# Autodesk Inventor assembly: BSHKSA6904ZZ-40_right
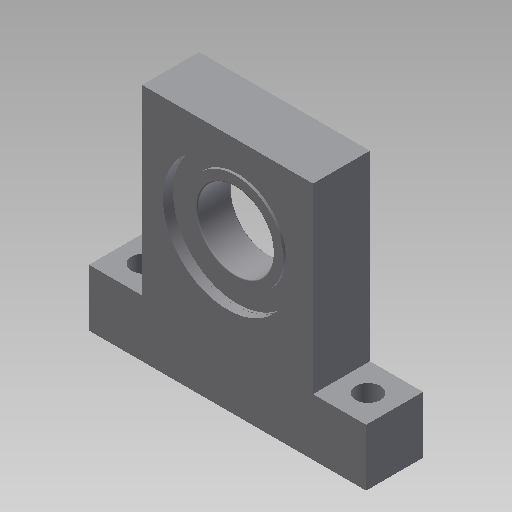
[picture p0: Inventor's stored thumbnail of the model, 512x512]
Saved by Autodesk Inventor 2021.2 (Build 252289000, 289)
## iProperties
Category: PARTsolutions
Company: MISUMI
Part Number: BSHKSA6904ZZ-40_right
Catalog Web Link: www.cadenas.de
Description: BSHKB, BSHK, BSHKA, BSHKSA, BSHFB, BSHF-Bearings with Housings - with Positioning Groove - T-Shaped - Base Face Type
Vendor: MISUMI
Document SubType Name: Assembly
Designer: gisen
Manufacturer: MISUMI
Mass: 38.5292 g
Surface Area: 155.893 cm^2
Volume: 38.5292 cm^3
Density: 1 g/cm^3
Title: BSHKSA6904ZZ-40
Author: Cadenas PARTsolutions
Comments: Bearings with Housings - with Positioning Groove - T-Shaped - Base Face Type
PSOL_IDENT_0: {$CADENAS_DATA\23d-libs\misumi\metric\12_bearing_holders\bshkb_asmtab.prj},259 {VTYP=3D},{STYP=ASSTA
PSOL_IDENT_1: B},{NB=BSHKSA6904ZZ-40},{LINA=BSHKSA6904ZZ-40},{NN=BSHKB, BSHK, BSHKA, BSHKSA, BSHFB, BSHF},{DATE=03
PSOL_IDENT_2: .06.2021 05:36:04},{GEOMDATE=10.09.2019 05:26:06},{VERSION=},{LINEID=210},{WBVAR=TS,MATB,MATH,STH,SE
PSOL_IDENT_3: AL,HH,ALT1,ALT2,ALT3},{WBNUMERIC=HH}  {NB=BSHKSA6904ZZ-40},{LINA=BSHKSA6904ZZ-40},{KT=DUMMY},{PN=BSH
PSOL_IDENT_4: KSA6904ZZ-40},{TYPE=BSHKSA},{TS=HS},{TSALG= 'HS', 'Height h Selectable', 'HC', 'Height h Specified'
PSOL_IDENT_5: },{MATB=SST},{MATBALG= 'ST','Steel','SST','Stainless Steel' },{MATH=A2000},{MATH1= 'A2000','2017 Alu
PSOL_IDENT_6: minum Alloy' },{STH=CA},{STH1=   'CA','Clear Anodizing'     },{ARR=304 Stainless Steel},{BN=6904},{B
PSOL_IDENT_7: N2=6904},{SEAL=ZZ},{SEALALG= 'ZZ', 'ZZ(Double Shielded)', 'VV', 'VV(Non-contact Rubber Seal)', 'DD'
PSOL_IDENT_8: , 'DD(Contact Rubber Seal)' },{HH=40},{HH1=40,50,60},{HH2=[30:80/1]},{DD=20},{D=37},{D3=39.800},{BT=
PSOL_IDENT_9: 1.600},{DDHH=34},{B=9},{H=63},{HD1=23},{L=73},{L1=59},{L2=45},{L3=36.5},{T=15},{S=15},{DD1=6.5},{TEM
PSOL_IDENT_10: P1=2},{NR=},{HHALG=40,50,60},{ALT1=},{ALT1ALG= '', 'Bearing and Retaining Ring Assembled', 'NA'  , '
PSOL_IDENT_11: with NA (Bearing and Retaining Ring not Assembled)'},{ALT1PN=},{ALT2=},{ALT2ALG='', 'w/o Chamfering'
PSOL_IDENT_12: , 'KCC', 'with KCC (C2 Chamfering)'},{ALT2PN=},{BNHALG=2},{ALT3=},{ALT3ALG= '','Not applicable' },{A
PSOL_IDENT_13: LT3PN=},{KKC=10},{PPATH=bshkb/bshkb_temp.prj}
NB: BSHKSA6904ZZ-40
NN: BSHKB, BSHK, BSHKA, BSHKSA, BSHFB, BSHF
NT: Bearings with Housings - with Positioning Groove - T-Shaped - Base Face Type
NBSYN: $PN.
LINA: BSHKSA6904ZZ-40
CATALOG: Misumi
PN: BSHKSA6904ZZ-40
TS: Height h Selectable
MATB: Stainless Steel
MATH: 2017 Aluminum Alloy
STH: Clear Anodizing
ARR: 304 Stainless Steel
BN: 6904
SEAL: ZZ(Double Shielded)
HH: 40
DD: 20
D: 37
DDHH: 34
B: 9
H: 63
L: 73
L1: 59
L2: 45
L3: 36.5
T: 15
S: 15
DD1: 6.5
ALT1: Bearing and Retaining Ring Assembled
ALT2: w/o Chamfering
ALT3: Not applicable
SUPPLIER: MISUMI
ARTICLENO: BSHKSA6904ZZ-40
BOMINFO: BSHKSA6904ZZ-40
CREATOR: CADENAS GmbH
## Documents named in this file (4)
- C:\Users\gisen\workspace\beetle_inventor_model\suspension\BSHKSA6904ZZ-40\BSHKSA6904ZZ-40_right.iam
- C:\Users\gisen\workspace\beetle_inventor_model\suspension\BSHKSA6904ZZ-40\BSHKSA6904ZZ-40_h_right.ipt
- C:\Users\gisen\workspace\beetle_inventor_model\suspension\BSHKSA6904ZZ-40\bearing_6904_right.ipt
- C:\Users\gisen\workspace\beetle_inventor_model\suspension\BSHKSA6904ZZ-40\RRING-C-INT-37_right.ipt
## Components (3 placed, 1 different names)
1. Part1:1 — to_bearing_Z@1 <-> to_housing_Z@2, to_bearing_XY@1 <-> to_housing_XY@2, to_rring_Z@1 <-> rr_Z@3, to_rring_XY@1 <-> rr_XY@3, to_bearing_YZ@1 <-> to_housing_YZ@2, to_rring_YZ@1 <-> rr_YZ@3
2. Part1:2 — to_bearing_Z@1 <-> to_housing_Z@2, to_bearing_XY@1 <-> to_housing_XY@2, to_bearing_YZ@1 <-> to_housing_YZ@2
3. Part1:3 — to_rring_Z@1 <-> rr_Z@3, to_rring_XY@1 <-> rr_XY@3, to_rring_YZ@1 <-> rr_YZ@3
## Relationships (6: Mate 4, Angle 2)
- to_bearing_Z@1 <-> to_housing_Z@2 [Mate]: Part1:1 ↔ Part1:2
- to_bearing_XY@1 <-> to_housing_XY@2 [Mate] (-9 mm): Part1:1 ↔ Part1:2
- to_rring_Z@1 <-> rr_Z@3 [Mate]: Part1:1 ↔ Part1:3
- to_rring_XY@1 <-> rr_XY@3 [Mate]: Part1:1 ↔ Part1:3
- to_bearing_YZ@1 <-> to_housing_YZ@2 [Angle] (0 deg): Part1:1 ↔ Part1:2
- to_rring_YZ@1 <-> rr_YZ@3 [Angle] (0 deg): Part1:1 ↔ Part1:3
